# Autodesk Inventor assembly: end effector worm gear 2
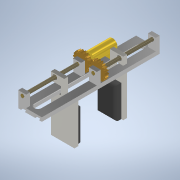
[picture p0: Inventor's stored thumbnail of the model, 180x180]
Saved by Autodesk Inventor 2021 (Build 250183000, 183)
## iProperties
Created: 2020-07-02
Part Number: end effector worm gear 2
Document SubType Name: Assembly
Designer: Ashiqrahman
Author: Ashiqrahman
## Documents named in this file (11)
- D:\projects\Intelligent Picking\my models\end effector worm gear 2\end effector worm gear 2.iam
- D:\projects\Intelligent Picking\my models\end effector worm gear 2\base plate.ipt
- D:\projects\Intelligent Picking\my models\end effector worm gear 2\lead screw.ipt
- D:\projects\Intelligent Picking\my models\end effector worm gear 2\lead screw 160.ipt
- D:\projects\Intelligent Picking\my models\end effector worm gear 2\Design Accelerator\Spur Gears2.iam
- D:\projects\Intelligent Picking\my models\end effector worm gear 2\jaws.ipt
- D:\projects\Intelligent Picking\my models\end effector worm gear 2\motor jaws.ipt
- D:\projects\Intelligent Picking\my models\end effector worm gear 2\rubber padding.ipt
- D:\projects\Intelligent Picking\my models\end effector worm gear 2\end_effector_clamp.ipt
- D:\projects\Intelligent Picking\my models\end effector worm gear 2\motor_casing.ipt
- D:\projects\Intelligent Picking\my models\end effector worm gear 2\motor_1.0.ipt
## Components (12 placed, 10 different names)
1. base plate:1 — Mate:1, Flush:1, Mate:2, Flush:2, Flush:3, Mate:8, Flush:14, Flush:17, Mate:14, Flush:18
2. lead screw:1 — Mate:2, Flush:2, Mate:3, Mate:5, Mate:7, Rotation/Translation:2
3. lead screw 160:1 — Mate:1, Flush:1, Mate:4, Mate:6, Rotation/Translation:1, Flush:4
4. Spur Gears:2 [sub-assembly] — Mate:3, Mate:4, Flush:3, Mate:5, Mate:6
5. jaws:1 — Rotation/Translation:1, Mate:10, Flush:12, Flush:13
6. jaws:2 — Mate:7, Mate:8, Rotation/Translation:2, Flush:5, Mate:9, Flush:6, Flush:7
7. motor jaws:1 — Flush:4
8. rubber padding:1 — Flush:5, Mate:9, Flush:6, Flush:7
9. rubber padding:2 — Mate:10, Flush:12, Flush:13
10. end_effector_clamp:1 — Flush:14, Flush:15, Flush:16, Rotation:1, Flush:17, Mate:14, Flush:18
11. motor_casing:1 — Flush:15, Flush:16, Mate:12, Mate:13, Mate:15
12. motor_1.0:1 — Mate:12, Mate:13, Rotation:1
## Relationships (31: Mate 14, Flush 14, RelateRotateTranslate 2, RelateRotation 1)
- Mate:1: base plate:1 ↔ lead screw 160:1
- Flush:1: base plate:1 ↔ lead screw 160:1
- Mate:2: base plate:1 ↔ lead screw:1
- Flush:2: base plate:1 ↔ lead screw:1
- Mate:3: lead screw:1 ↔ Spur Gears:2
- Mate:4: lead screw 160:1 ↔ Spur Gears:2
- Flush:3 (11 mm): base plate:1 ↔ Spur Gears:2
- Mate:5: lead screw:1 ↔ Spur Gears:2
- Mate:6: lead screw 160:1 ↔ Spur Gears:2
- Mate:7: lead screw:1 ↔ jaws:2
- Mate:8: base plate:1 ↔ jaws:2
- Rotation/Translation:1 [RelateRotateTranslate] (25.133 mm): lead screw 160:1 ↔ jaws:1
- Rotation/Translation:2 [RelateRotateTranslate] (25.133 mm): lead screw:1 ↔ jaws:2
- Flush:4: lead screw 160:1 ↔ motor jaws:1
- Flush:5: jaws:2 ↔ rubber padding:1
- Mate:9: jaws:2 ↔ rubber padding:1
- Flush:6 (5 mm): jaws:2 ↔ rubber padding:1
- Flush:7: jaws:2 ↔ rubber padding:1
- Mate:10: jaws:1 ↔ rubber padding:2
- Flush:12: jaws:1 ↔ rubber padding:2
- Flush:13 (5 mm): jaws:1 ↔ rubber padding:2
- Flush:14: base plate:1 ↔ end_effector_clamp:1
- Flush:15: end_effector_clamp:1 ↔ motor_casing:1
- Flush:16: end_effector_clamp:1 ↔ motor_casing:1
- Mate:12: motor_casing:1 ↔ motor_1.0:1
- Mate:13: motor_casing:1 ↔ motor_1.0:1
- Rotation:1 [RelateRotation] (1 ul): end_effector_clamp:1 ↔ motor_1.0:1
- Flush:17: base plate:1 ↔ end_effector_clamp:1
- Mate:14: base plate:1 ↔ end_effector_clamp:1
- Flush:18 (100 mm): base plate:1 ↔ end_effector_clamp:1
- Mate:15: motor_casing:1
